# Autodesk Inventor assembly: Ensamble
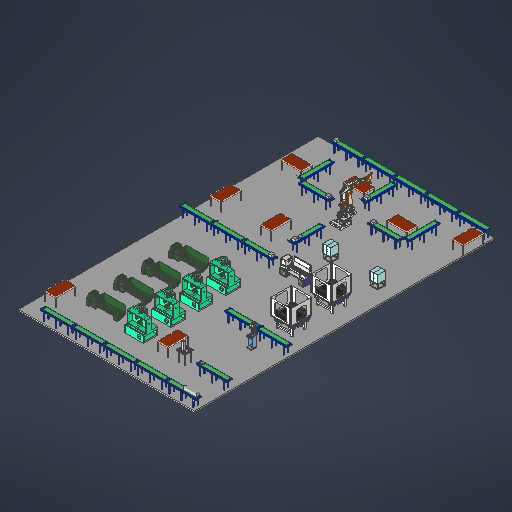
[picture p0: Inventor's stored thumbnail of the model, 512x512]
Saved by Autodesk Inventor 2026.2 (Build 302298000, 298)
## iProperties
Created: 2025-11-25
Part Number: Ensamble
Document SubType Name: Assembly
Designer: USUARIO
Author: USUARIO
## Documents named in this file (16)
- F:\UNAL\14. SEMESTRE\AUTOMATIZACIÓN DE PROCESOS DE MANUFACTURA\GitHub\Los4Automaticos\CAD\InventorProyecto\Ensamble.iam
- F:\UNAL\14. SEMESTRE\AUTOMATIZACIÓN DE PROCESOS DE MANUFACTURA\GitHub\Los4Automaticos\CAD\InventorProyecto\Floor.ipt
- F:\UNAL\14. SEMESTRE\AUTOMATIZACIÓN DE PROCESOS DE MANUFACTURA\GitHub\Los4Automaticos\CAD\InventorProyecto\Talladora.ipt
- F:\UNAL\14. SEMESTRE\AUTOMATIZACIÓN DE PROCESOS DE MANUFACTURA\GitHub\Los4Automaticos\CAD\InventorProyecto\Torno1.ipt
- F:\UNAL\14. SEMESTRE\AUTOMATIZACIÓN DE PROCESOS DE MANUFACTURA\GitHub\Los4Automaticos\CAD\InventorProyecto\Torno2.ipt
- F:\UNAL\14. SEMESTRE\AUTOMATIZACIÓN DE PROCESOS DE MANUFACTURA\GitHub\Los4Automaticos\CAD\InventorProyecto\FresadoraGrande.ipt
- F:\UNAL\14. SEMESTRE\AUTOMATIZACIÓN DE PROCESOS DE MANUFACTURA\GitHub\Los4Automaticos\CAD\InventorProyecto\FresadoraPequeña.ipt
- F:\UNAL\14. SEMESTRE\AUTOMATIZACIÓN DE PROCESOS DE MANUFACTURA\GitHub\Los4Automaticos\CAD\InventorProyecto\Taladro.ipt
- F:\UNAL\14. SEMESTRE\AUTOMATIZACIÓN DE PROCESOS DE MANUFACTURA\GitHub\Los4Automaticos\CAD\InventorProyecto\Verificadora.ipt
- F:\UNAL\14. SEMESTRE\AUTOMATIZACIÓN DE PROCESOS DE MANUFACTURA\GitHub\Los4Automaticos\CAD\InventorProyecto\Robot.ipt
- F:\UNAL\14. SEMESTRE\AUTOMATIZACIÓN DE PROCESOS DE MANUFACTURA\GitHub\Los4Automaticos\CAD\InventorProyecto\Gripper.ipt
- F:\UNAL\14. SEMESTRE\AUTOMATIZACIÓN DE PROCESOS DE MANUFACTURA\GitHub\Los4Automaticos\CAD\InventorProyecto\MesaEnsamble.iam
- F:\UNAL\14. SEMESTRE\AUTOMATIZACIÓN DE PROCESOS DE MANUFACTURA\GitHub\Los4Automaticos\CAD\InventorProyecto\Banda.iam
- F:\UNAL\14. SEMESTRE\AUTOMATIZACIÓN DE PROCESOS DE MANUFACTURA\GitHub\Los4Automaticos\CAD\InventorProyecto\Material.ipt
- F:\UNAL\14. SEMESTRE\AUTOMATIZACIÓN DE PROCESOS DE MANUFACTURA\GitHub\Los4Automaticos\CAD\InventorProyecto\Carcasa.ipt
- F:\UNAL\14. SEMESTRE\AUTOMATIZACIÓN DE PROCESOS DE MANUFACTURA\GitHub\Los4Automaticos\CAD\InventorProyecto\Circulo.ipt
## Components (57 placed, 15 different names)
1. Floor:1 — Coincidencia:7, Coincidencia:8, Coincidencia:9, Coincidencia:11, Coincidencia:12, Coincidencia:14, Coincidencia:15, Coincidencia:16, Coincidencia:24, Coincidencia:25, Coincidencia:26, Coincidencia:27, Coincidencia:28, Coincidencia:29, Coincidencia:30, Coincidencia:31, Coincidencia:32, Coincidencia:33, Coincidencia:34, Coincidencia:35, Coincidencia:36, Coincidencia:37, Coincidencia:38, Coincidencia:39, Coincidencia:40, Coincidencia:41, Coincidencia:42, Coincidencia:43, Coincidencia:44, Coincidencia:45, Coincidencia:46, Coincidencia:47, Coincidencia:48, Coincidencia:49, Coincidencia:50, Coincidencia:51, Coincidencia:52, Coincidencia:53, Nivelación:5, Tangente:1, Coincidencia:59, Coincidencia:60, Coincidencia:61, Nivelación:18, Nivelación:19, Tangente:3, Coincidencia:76, Coincidencia:80, Coincidencia:82, Coincidencia:84, Coincidencia:90, Nivelación:47, Nivelación:55, Nivelación:56, Nivelación:57, Nivelación:58, Tangente:4, Tangente:5
2. Torno1:1 — Coincidencia:14, Nivelación:29, Nivelación:30, Coincidencia:74, Coincidencia:75
3. Torno2:1 — Coincidencia:25, Nivelación:7, Nivelación:9, Coincidencia:62, Nivelación:14
4. Torno2:2 — Coincidencia:24, Nivelación:10, Nivelación:16
5. FresadoraGrande:1 — Coincidencia:16, Nivelación:18, Coincidencia:66, Nivelación:28
6. FresadoraGrande:2 — Coincidencia:15, Nivelación:19, Coincidencia:66, Nivelación:27, Coincidencia:73, Nivelación:29, Coincidencia:74
7. FresadoraPequeña:1 — Coincidencia:12, Coincidencia:72, Nivelación:26
8. Taladro:1 — Coincidencia:11, Nivelación:23, Coincidencia:71, Nivelación:24
9. Verificadora:1 — Coincidencia:8, Nivelación:27, Coincidencia:73, Nivelación:33, Coincidencia:86
10. Verificadora:2 — Coincidencia:7, Nivelación:33, Coincidencia:86, Coincidencia:87
11. Robot:1 — Coincidencia:9, Insertar:1, Coincidencia:88, Nivelación:36, Coincidencia:92, Nivelación:39, Coincidencia:94
12. Gripper:1 — Insertar:1
13. Talladora:1 — Coincidencia:29, Nivelación:11, Coincidencia:63, Nivelación:17, Nivelación:28
14. Talladora:2 — Coincidencia:28, Nivelación:11, Nivelación:12, Coincidencia:63, Coincidencia:64, Nivelación:16, Nivelación:25
15. Talladora:3 — Coincidencia:27, Nivelación:12, Nivelación:13, Coincidencia:64, Coincidencia:65, Nivelación:15
16. Talladora:4 — Coincidencia:26, Coincidencia:62, Nivelación:13, Coincidencia:65, Nivelación:14, Coincidencia:69, Nivelación:21, Coincidencia:115
17. MesaEnsamble:1 [sub-assembly] — Coincidencia:35, Nivelación:32, Coincidencia:81, Nivelación:34, Coincidencia:85
18. MesaEnsamble:2 [sub-assembly] — Coincidencia:36, Coincidencia:58, Nivelación:6, Nivelación:32
19. MesaEnsamble:3 [sub-assembly] — Coincidencia:34, Nivelación:21, Nivelación:23, Coincidencia:71, Coincidencia:115
20. MesaEnsamble:4 [sub-assembly] — Coincidencia:33, Nivelación:53, Coincidencia:105
21. MesaEnsamble:5 [sub-assembly] — Coincidencia:32, Nivelación:52, Coincidencia:104
22. MesaEnsamble:6 [sub-assembly] — Coincidencia:31, Nivelación:54, Coincidencia:106
23. MesaEnsamble:7 [sub-assembly] — Coincidencia:30, Nivelación:55, Coincidencia:107
24. Banda:1 [sub-assembly] — Coincidencia:37, Coincidencia:54, Nivelación:1, Tangente:1
25. Banda:2 [sub-assembly] — Coincidencia:38, Coincidencia:54, Coincidencia:55, Nivelación:1, Nivelación:2
26. Banda:3 [sub-assembly] — Coincidencia:39, Coincidencia:55, Nivelación:2, Nivelación:3, Coincidencia:56, Coincidencia:69
27. Banda:4 [sub-assembly] — Coincidencia:40, Nivelación:3, Coincidencia:56, Nivelación:4, Coincidencia:57
28. Banda:5 [sub-assembly] — Coincidencia:41, Nivelación:4, Coincidencia:57, Nivelación:5, Coincidencia:58, Nivelación:6
29. Banda:6 [sub-assembly] — Coincidencia:43, Coincidencia:67, Nivelación:20, Nivelación:26, Nivelación:56
30. Banda:7 [sub-assembly] — Coincidencia:42, Tangente:3, Nivelación:24, Coincidencia:116, Tangente:22, Tangente:23
31. Banda:8 [sub-assembly] — Coincidencia:44, Nivelación:30, Coincidencia:75, Coincidencia:77, Nivelación:31, Coincidencia:109, Nivelación:59, Tangente:13
32. Banda:9 [sub-assembly] — Coincidencia:48, Nivelación:41, Coincidencia:94, Coincidencia:101, Coincidencia:102, Coincidencia:112, Nivelación:63, Tangente:19
33. Banda:10 [sub-assembly] — Coincidencia:47, Coincidencia:95, Nivelación:43, Nivelación:47, Coincidencia:107, Nivelación:57
34. Banda:11 [sub-assembly] — Coincidencia:53, Nivelación:37, Coincidencia:89, Nivelación:53, Coincidencia:105, Coincidencia:114, Nivelación:65, Tangente:21
35. Banda:12 [sub-assembly] — Coincidencia:46, Coincidencia:95, Nivelación:43, Coincidencia:96, Nivelación:44
36. Banda:13 [sub-assembly] — Coincidencia:45, Coincidencia:96, Nivelación:44, Coincidencia:97, Nivelación:45
37. Banda:14 [sub-assembly] — Coincidencia:49, Coincidencia:98, Nivelación:46, Coincidencia:111, Nivelación:62, Tangente:18
38. Banda:15 [sub-assembly] — Coincidencia:50, Coincidencia:101, Coincidencia:102, Nivelación:54, Coincidencia:106
39. Banda:16 [sub-assembly] — Coincidencia:51, Coincidencia:99, Coincidencia:100, Nivelación:52, Coincidencia:104
40. Banda:17 [sub-assembly] — Coincidencia:52, Coincidencia:92, Nivelación:39, Nivelación:41, Coincidencia:99, Coincidencia:100, Coincidencia:113, Nivelación:64, Tangente:20
41. Torno2:3 — Coincidencia:60, Nivelación:8, Nivelación:9, Nivelación:10, Nivelación:17
42. Torno2:4 — Coincidencia:59, Nivelación:7, Nivelación:8, Nivelación:15
43. Banda:18 [sub-assembly] — Coincidencia:61, Coincidencia:67, Nivelación:20, Coincidencia:72, Nivelación:25
44. Banda:19 [sub-assembly] — Coincidencia:76, Coincidencia:77, Nivelación:31, Coincidencia:81, Coincidencia:83, Nivelación:48
45. Banda:20 [sub-assembly] — Coincidencia:80, Coincidencia:87, Nivelación:35, Coincidencia:88, Nivelación:36, Nivelación:37, Coincidencia:89, Nivelación:60, Nivelación:61, Tangente:14, Coincidencia:117, Tangente:24
46. Banda:21 [sub-assembly] — Coincidencia:90, Coincidencia:97, Nivelación:45, Coincidencia:98, Nivelación:46
47. MesaEnsamble:8 [sub-assembly] — Coincidencia:84, Nivelación:34, Coincidencia:85, Nivelación:35
48. Banda:22 [sub-assembly] — Coincidencia:82, Coincidencia:83, Nivelación:48
49. Material:1 — Nivelación:58, Tangente:4, Tangente:5
50. Carcasa:1 — Coincidencia:109, Nivelación:59, Tangente:13
51. Carcasa:2 — Nivelación:60, Nivelación:61, Tangente:14, Tangente:25
52. Carcasa:3 — Coincidencia:111, Nivelación:62, Tangente:18
53. Carcasa:4 — Coincidencia:112, Nivelación:63, Tangente:19
54. Carcasa:5 — Coincidencia:113, Nivelación:64, Tangente:20
55. Carcasa:6 — Coincidencia:114, Nivelación:65, Tangente:21
56. Circulo:1 — Coincidencia:116, Tangente:22, Tangente:23
57. Circulo:2 — Coincidencia:117, Tangente:24, Tangente:25
## Relationships (166: Mate 93, Flush 58, Tangent 14, Insert 1)
- Coincidencia:7 [Mate]: Floor:1 ↔ Verificadora:2
- Coincidencia:8 [Mate]: Floor:1 ↔ Verificadora:1
- Coincidencia:9 [Mate]: Floor:1 ↔ Robot:1
- Coincidencia:11 [Mate]: Floor:1 ↔ Taladro:1
- Coincidencia:12 [Mate]: Floor:1 ↔ FresadoraPequeña:1
- Coincidencia:14 [Mate]: Floor:1 ↔ Torno1:1
- Coincidencia:15 [Mate]: Floor:1 ↔ FresadoraGrande:2
- Coincidencia:16 [Mate]: Floor:1 ↔ FresadoraGrande:1
- Insertar:1: Robot:1 ↔ Gripper:1
- Coincidencia:24 [Mate]: Floor:1 ↔ Torno2:2
- Coincidencia:25 [Mate]: Floor:1 ↔ Torno2:1
- Coincidencia:26 [Mate]: Floor:1 ↔ Talladora:4
- Coincidencia:27 [Mate]: Floor:1 ↔ Talladora:3
- Coincidencia:28 [Mate]: Floor:1 ↔ Talladora:2
- Coincidencia:29 [Mate]: Floor:1 ↔ Talladora:1
- Coincidencia:30 [Mate]: Floor:1 ↔ MesaEnsamble:7
- Coincidencia:31 [Mate]: Floor:1 ↔ MesaEnsamble:6
- Coincidencia:32 [Mate]: Floor:1 ↔ MesaEnsamble:5
- Coincidencia:33 [Mate]: Floor:1 ↔ MesaEnsamble:4
- Coincidencia:34 [Mate]: Floor:1 ↔ MesaEnsamble:3
- Coincidencia:35 [Mate]: Floor:1 ↔ MesaEnsamble:1
- Coincidencia:36 [Mate]: Floor:1 ↔ MesaEnsamble:2
- Coincidencia:37 [Mate]: Floor:1 ↔ Banda:1
- Coincidencia:38 [Mate]: Floor:1 ↔ Banda:2
- Coincidencia:39 [Mate]: Floor:1 ↔ Banda:3
- Coincidencia:40 [Mate]: Floor:1 ↔ Banda:4
- Coincidencia:41 [Mate]: Floor:1 ↔ Banda:5
- Coincidencia:42 [Mate]: Floor:1 ↔ Banda:7
- Coincidencia:43 [Mate]: Floor:1 ↔ Banda:6
- Coincidencia:44 [Mate]: Floor:1 ↔ Banda:8
- Coincidencia:45 [Mate]: Floor:1 ↔ Banda:13
- Coincidencia:46 [Mate]: Floor:1 ↔ Banda:12
- Coincidencia:47 [Mate]: Floor:1 ↔ Banda:10
- Coincidencia:48 [Mate]: Floor:1 ↔ Banda:9
- Coincidencia:49 [Mate]: Floor:1 ↔ Banda:14
- Coincidencia:50 [Mate]: Floor:1 ↔ Banda:15
- Coincidencia:51 [Mate]: Floor:1 ↔ Banda:16
- Coincidencia:52 [Mate]: Floor:1 ↔ Banda:17
- Coincidencia:53 [Mate]: Floor:1 ↔ Banda:11
- Coincidencia:54 [Mate]: Banda:1 ↔ Banda:2
- Coincidencia:55 [Mate]: Banda:2 ↔ Banda:3
- Nivelación:1 [Flush]: Banda:1 ↔ Banda:2
- Nivelación:2 [Flush]: Banda:2 ↔ Banda:3
- Nivelación:3 [Flush]: Banda:3 ↔ Banda:4
- Coincidencia:56 [Mate]: Banda:3 ↔ Banda:4
- Nivelación:4 [Flush]: Banda:4 ↔ Banda:5
- Coincidencia:57 [Mate]: Banda:4 ↔ Banda:5
- Nivelación:5 [Flush]: Floor:1 ↔ Banda:5
- Tangente:1: Floor:1 ↔ Banda:1
- Coincidencia:58 [Mate] (1000 mm): MesaEnsamble:2 ↔ Banda:5
- Nivelación:6 [Flush] (-1000 mm): MesaEnsamble:2 ↔ Banda:5
- Coincidencia:59 [Mate]: Floor:1 ↔ Torno2:4
- Coincidencia:60 [Mate]: Floor:1 ↔ Torno2:3
- Coincidencia:61 [Mate]: Floor:1 ↔ Banda:18
- Nivelación:7 [Flush]: Torno2:1 ↔ Torno2:4
- Nivelación:8 [Flush]: Torno2:3 ↔ Torno2:4
- Nivelación:9 [Flush]: Torno2:1 ↔ Torno2:3
- Nivelación:10 [Flush]: Torno2:2 ↔ Torno2:3
- Coincidencia:62 [Mate] (1000 mm): Torno2:1 ↔ Talladora:4
- Nivelación:11 [Flush]: Talladora:1 ↔ Talladora:2
- Nivelación:12 [Flush]: Talladora:2 ↔ Talladora:3
- Nivelación:13 [Flush]: Talladora:3 ↔ Talladora:4
- Coincidencia:63 [Mate] (1000 mm): Talladora:1 ↔ Talladora:2
- Coincidencia:64 [Mate] (1000 mm): Talladora:2 ↔ Talladora:3
- Coincidencia:65 [Mate] (1000 mm): Talladora:3 ↔ Talladora:4
- Nivelación:14 [Flush]: Torno2:1 ↔ Talladora:4
- Nivelación:15 [Flush]: Talladora:3 ↔ Torno2:4
- Nivelación:16 [Flush]: Torno2:2 ↔ Talladora:2
- Nivelación:17 [Flush]: Talladora:1 ↔ Torno2:3
- Nivelación:18 [Flush] (1000 mm): Floor:1 ↔ FresadoraGrande:1
- Nivelación:19 [Flush] (1000 mm): Floor:1 ↔ FresadoraGrande:2
- Coincidencia:66 [Mate] (1500 mm): FresadoraGrande:1 ↔ FresadoraGrande:2
- Coincidencia:67 [Mate]: Banda:6 ↔ Banda:18
- Nivelación:20 [Flush]: Banda:6 ↔ Banda:18
- Coincidencia:69 [Mate] (2000 mm): Talladora:4 ↔ Banda:3
- Nivelación:21 [Flush]: Talladora:4 ↔ MesaEnsamble:3
- Nivelación:23 [Flush]: Taladro:1 ↔ MesaEnsamble:3
- Coincidencia:71 [Mate] (600 mm): Taladro:1 ↔ MesaEnsamble:3
- Coincidencia:72 [Mate] (500 mm): FresadoraPequeña:1 ↔ Banda:18
- Tangente:3: Floor:1 ↔ Banda:7
- Nivelación:24 [Flush]: Taladro:1 ↔ Banda:7
- Nivelación:25 [Flush] (375 mm): Talladora:2 ↔ Banda:18
- Nivelación:26 [Flush] (200 mm): FresadoraPequeña:1 ↔ Banda:6
- Nivelación:27 [Flush]: FresadoraGrande:2 ↔ Verificadora:1
- Coincidencia:73 [Mate] (2000 mm): FresadoraGrande:2 ↔ Verificadora:1
- Nivelación:28 [Flush]: FresadoraGrande:1 ↔ Talladora:1
- Nivelación:29 [Flush]: Torno1:1 ↔ FresadoraGrande:2
- Nivelación:30 [Flush]: Torno1:1 ↔ Banda:8
- Coincidencia:74 [Mate] (1500 mm): Torno1:1 ↔ FresadoraGrande:2
- Coincidencia:75 [Mate] (500 mm): Torno1:1 ↔ Banda:8
- Coincidencia:76 [Mate]: Floor:1 ↔ Banda:19
- Coincidencia:77 [Mate]: Banda:8 ↔ Banda:19
- Nivelación:31 [Flush]: Banda:8 ↔ Banda:19
- Nivelación:32 [Flush]: MesaEnsamble:1 ↔ MesaEnsamble:2
- Nivelación:33 [Flush]: Verificadora:1 ↔ Verificadora:2
- Coincidencia:80 [Mate]: Floor:1 ↔ Banda:20
- Coincidencia:81 [Mate] (1500 mm): MesaEnsamble:1 ↔ Banda:19
- Coincidencia:82 [Mate]: Floor:1 ↔ Banda:22
- Coincidencia:83 [Mate]: Banda:19 ↔ Banda:22
- Coincidencia:84 [Mate]: Floor:1 ↔ MesaEnsamble:8
- Nivelación:34 [Flush]: MesaEnsamble:1 ↔ MesaEnsamble:8
- Coincidencia:85 [Mate] (3000 mm): MesaEnsamble:1 ↔ MesaEnsamble:8
- Coincidencia:86 [Mate] (3000 mm): Verificadora:1 ↔ Verificadora:2
- Coincidencia:87 [Mate] (1383.75 mm): Verificadora:2 ↔ Banda:20
- Nivelación:35 [Flush]: Banda:20 ↔ MesaEnsamble:8
- Coincidencia:88 [Mate] (1000 mm): Robot:1 ↔ Banda:20
- Nivelación:36 [Flush] (-412 mm): Robot:1 ↔ Banda:20
- Nivelación:37 [Flush]: Banda:11 ↔ Banda:20
- Coincidencia:89 [Mate] (3129 mm): Banda:11 ↔ Banda:20
- Coincidencia:90 [Mate]: Floor:1 ↔ Banda:21
- Coincidencia:92 [Mate] (700 mm): Robot:1 ↔ Banda:17
- Nivelación:39 [Flush]: Robot:1 ↔ Banda:17
- Nivelación:41 [Flush]: Banda:9 ↔ Banda:17
- Coincidencia:94 [Mate] (1000 mm): Robot:1 ↔ Banda:9
- Coincidencia:95 [Mate]: Banda:10 ↔ Banda:12
- Nivelación:43 [Flush]: Banda:10 ↔ Banda:12
- Coincidencia:96 [Mate]: Banda:12 ↔ Banda:13
- Nivelación:44 [Flush]: Banda:12 ↔ Banda:13
- Coincidencia:97 [Mate]: Banda:13 ↔ Banda:21
- Nivelación:45 [Flush]: Banda:13 ↔ Banda:21
- Coincidencia:98 [Mate]: Banda:14 ↔ Banda:21
- Nivelación:46 [Flush]: Banda:14 ↔ Banda:21
- Nivelación:47 [Flush]: Floor:1 ↔ Banda:10
- Nivelación:48 [Flush]: Banda:19 ↔ Banda:22
- Coincidencia:99 [Mate] (30 mm): Banda:16 ↔ Banda:17
- Coincidencia:100 [Mate] (30 mm): Banda:16 ↔ Banda:17
- Coincidencia:101 [Mate] (30 mm): Banda:9 ↔ Banda:15
- Coincidencia:102 [Mate] (30 mm): Banda:9 ↔ Banda:15
- Nivelación:52 [Flush] (500 mm): MesaEnsamble:5 ↔ Banda:16
- Coincidencia:104 [Mate] (300 mm): MesaEnsamble:5 ↔ Banda:16
- Nivelación:53 [Flush] (500 mm): MesaEnsamble:4 ↔ Banda:11
- Coincidencia:105 [Mate] (300 mm): MesaEnsamble:4 ↔ Banda:11
- Nivelación:54 [Flush] (500 mm): MesaEnsamble:6 ↔ Banda:15
- Coincidencia:106 [Mate] (300 mm): MesaEnsamble:6 ↔ Banda:15
- Nivelación:55 [Flush]: Floor:1 ↔ MesaEnsamble:7
- Coincidencia:107 [Mate] (300 mm): MesaEnsamble:7 ↔ Banda:10
- Nivelación:56 [Flush]: Floor:1 ↔ Banda:6
- Nivelación:57 [Flush]: Floor:1 ↔ Banda:10
- Nivelación:58 [Flush] (100 mm): Floor:1 ↔ Material:1
- Tangente:4 (235 mm): Floor:1 ↔ Material:1
- Tangente:5 (733 mm): Floor:1 ↔ Material:1
- Coincidencia:109 [Mate]: Banda:8 ↔ Carcasa:1
- Nivelación:59 [Flush] (-20 mm): Banda:8 ↔ Carcasa:1
- Tangente:13 (-150 mm): Banda:8 ↔ Carcasa:1
- Nivelación:60 [Flush] (-150 mm): Banda:20 ↔ Carcasa:2
- Nivelación:61 [Flush] (20 mm): Banda:20 ↔ Carcasa:2
- Tangente:14 (-150 mm): Banda:20 ↔ Carcasa:2
- Coincidencia:111 [Mate]: Banda:14 ↔ Carcasa:3
- Nivelación:62 [Flush] (20 mm): Banda:14 ↔ Carcasa:3
- Tangente:18 (-150 mm): Banda:14 ↔ Carcasa:3
- Coincidencia:112 [Mate]: Banda:9 ↔ Carcasa:4
- Nivelación:63 [Flush] (20 mm): Banda:9 ↔ Carcasa:4
- Tangente:19 (-150 mm): Banda:9 ↔ Carcasa:4
- Coincidencia:113 [Mate]: Banda:17 ↔ Carcasa:5
- Nivelación:64 [Flush] (20 mm): Banda:17 ↔ Carcasa:5
- Tangente:20 (-150 mm): Banda:17 ↔ Carcasa:5
- Coincidencia:114 [Mate]: Banda:11 ↔ Carcasa:6
- Nivelación:65 [Flush] (20 mm): Banda:11 ↔ Carcasa:6
- Tangente:21 (-150 mm): Banda:11 ↔ Carcasa:6
- Coincidencia:115 [Mate] (1073.5 mm): Talladora:4 ↔ MesaEnsamble:3
- Coincidencia:116 [Mate]: Banda:7 ↔ Circulo:1
- Tangente:22 (-150 mm): Banda:7 ↔ Circulo:1
- Tangente:23 (20 mm): Banda:7 ↔ Circulo:1
- Coincidencia:117 [Mate]: Banda:20 ↔ Circulo:2
- Tangente:24 (20 mm): Banda:20 ↔ Circulo:2
- Tangente:25 (150 mm): Carcasa:2 ↔ Circulo:2
